# Autodesk Inventor assembly: tip_hl_ass_1
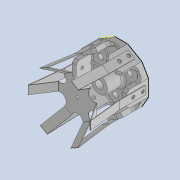
[picture p0: Inventor's stored thumbnail of the model, 180x180]
Saved by Autodesk Inventor 2020 (Build 240168000, 168)
## iProperties
Created: 2021-10-03
Part Number: tip_hl_ass_1
Document SubType Name: Assembly
Designer: Shuang Peng
Author: Shuang Peng
## Documents named in this file (6)
- D:\projects-3\torque fb tip\hardware\compact_ma_tmp\tip_hl_ass_1.iam
- D:\projects-3\torque fb tip\hardware\compact_ma_tmp\fin_12mm_h.ipt
- D:\projects-3\torque fb tip\hardware\compact_ma_tmp\fin_12mm.ipt
- D:\projects-3\torque fb tip\hardware\compact_ma_tmp\fin_8mm.ipt
- D:\projects-3\torque fb tip\hardware\compact_ma_tmp\mid_7mm.ipt
- D:\projects-3\torque fb tip\hardware\compact_ma_tmp\up_10mm_pr.ipt
## Components (20 placed, 5 different names)
1. fin_12mm_h:1 — Insert:11, Insert:29
2. fin_12mm_h:2 — Insert:12, Insert:28
3. fin_12mm_h:3 — Insert:7, Insert:27
4. fin_12mm_h:4 — Insert:10, Insert:30
5. fin_12mm_h:5 — Insert:9, Insert:26
6. fin_12mm_h:6 — Insert:8, Insert:25
7. fin_12mm:1 — Insert:8, Insert:14
8. fin_12mm:2 — Insert:9, Insert:15
9. fin_12mm:3 — Insert:10, Insert:16
10. fin_12mm:4 — Insert:12, Insert:18
11. fin_12mm:5 — Insert:11, Insert:17
12. fin_12mm:6 — Insert:7, Insert:13
13. fin_8mm:1 — Insert:13, Insert:22
14. fin_8mm:2 — Insert:15, Insert:24
15. fin_8mm:3 — Insert:14, Insert:21
16. fin_8mm:4 — Insert:18, Insert:23
17. fin_8mm:5 — Insert:16, Insert:20
18. fin_8mm:6 — Insert:17, Insert:19
19. mid_7mm:1 — Insert:19, Insert:20, Insert:21, Insert:22, Insert:23, Insert:24
20. up_10mm_pr:1 — Insert:25, Insert:26, Insert:27, Insert:28, Insert:29, Insert:30
## Relationships (24: Insert 24)
- Insert:7: fin_12mm_h:3 ↔ fin_12mm:6
- Insert:8: fin_12mm_h:6 ↔ fin_12mm:1
- Insert:9: fin_12mm_h:5 ↔ fin_12mm:2
- Insert:10: fin_12mm_h:4 ↔ fin_12mm:3
- Insert:11: fin_12mm_h:1 ↔ fin_12mm:5
- Insert:12: fin_12mm_h:2 ↔ fin_12mm:4
- Insert:13: fin_12mm:6 ↔ fin_8mm:1
- Insert:14: fin_12mm:1 ↔ fin_8mm:3
- Insert:15: fin_12mm:2 ↔ fin_8mm:2
- Insert:16: fin_12mm:3 ↔ fin_8mm:5
- Insert:17: fin_12mm:5 ↔ fin_8mm:6
- Insert:18: fin_12mm:4 ↔ fin_8mm:4
- Insert:19: fin_8mm:6 ↔ mid_7mm:1
- Insert:20: fin_8mm:5 ↔ mid_7mm:1
- Insert:21: fin_8mm:3 ↔ mid_7mm:1
- Insert:22: fin_8mm:1 ↔ mid_7mm:1
- Insert:23: fin_8mm:4 ↔ mid_7mm:1
- Insert:24: fin_8mm:2 ↔ mid_7mm:1
- Insert:25: fin_12mm_h:6 ↔ up_10mm_pr:1
- Insert:26: fin_12mm_h:5 ↔ up_10mm_pr:1
- Insert:27: fin_12mm_h:3 ↔ up_10mm_pr:1
- Insert:28: fin_12mm_h:2 ↔ up_10mm_pr:1
- Insert:29: fin_12mm_h:1 ↔ up_10mm_pr:1
- Insert:30: fin_12mm_h:4 ↔ up_10mm_pr:1
